# Autodesk Inventor assembly: Vibrometer Cover
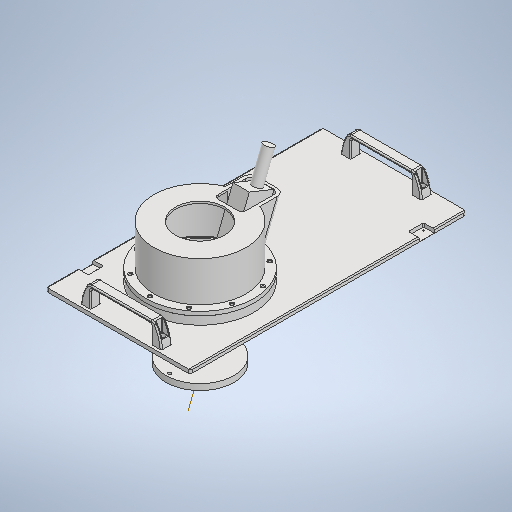
[picture p0: Inventor's stored thumbnail of the model, 512x512]
Saved by Autodesk Inventor 2026.2 (Build 302298000, 298)
## iProperties
Created: 2026-03-30
Part Number: Vibrometer Cover
Document SubType Name: Assembly
Designer: mumin
Author: mumin
## Documents named in this file (7)
- C:\GitHub\In-situ-monitoring-of-powder-bed-fusion-additive-manufacturing\system_development\Orichalcum\v0.4\Vibrometer Cover.iam
- C:\GitHub\In-situ-monitoring-of-powder-bed-fusion-additive-manufacturing\system_development\Orichalcum\v0.4\12mm Cover.ipt
- C:\GitHub\In-situ-monitoring-of-powder-bed-fusion-additive-manufacturing\system_development\Orichalcum\v0.4\Handle.ipt
- C:\GitHub\In-situ-monitoring-of-powder-bed-fusion-additive-manufacturing\system_development\Orichalcum\v0.4\SealedGlassRing.ipt
- C:\GitHub\In-situ-monitoring-of-powder-bed-fusion-additive-manufacturing\system_development\Orichalcum\v0.4\Vibrometer Housing.ipt
- C:\GitHub\In-situ-monitoring-of-powder-bed-fusion-additive-manufacturing\system_development\Orichalcum\v0.4\Build Plate.ipt
- C:\GitHub\In-situ-monitoring-of-powder-bed-fusion-additive-manufacturing\system_development\Orichalcum\v0.4\Updated Laser Scanner.ipt
## Components (7 placed, 6 different names)
1. 12mm Cover:1 — Insert:1, Insert:2, Insert:3, Insert:4, Insert:7
2. Handle:1 — Insert:1
3. Handle:2 — Insert:2
4. SealedGlassRing:1 — Insert:3, Insert:4, Insert:5, Insert:6
5. Vibrometer Housing:1 — Insert:5, Insert:6, Mate:1, Mate:2
6. Build Plate:1 — Insert:7
7. Updated Laser Scanner:1 — Mate:1, Mate:2
## Relationships (9: Insert 7, Mate 2)
- Insert:1: 12mm Cover:1 ↔ Handle:1
- Insert:2: 12mm Cover:1 ↔ Handle:2
- Insert:3: 12mm Cover:1 ↔ SealedGlassRing:1
- Insert:4: 12mm Cover:1 ↔ SealedGlassRing:1
- Insert:5: SealedGlassRing:1 ↔ Vibrometer Housing:1
- Insert:6: SealedGlassRing:1 ↔ Vibrometer Housing:1
- Insert:7 (150 mm): 12mm Cover:1 ↔ Build Plate:1
- Mate:1: Vibrometer Housing:1 ↔ Updated Laser Scanner:1
- Mate:2 (10 mm): Vibrometer Housing:1 ↔ Updated Laser Scanner:1
